# Autodesk Inventor assembly: Blue Alliance Bucket
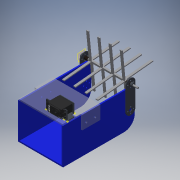
[picture p0: Inventor's stored thumbnail of the model, 180x180]
Saved by Autodesk Inventor 2016 (Build 200138000, 138)
## iProperties
Created: 2015-12-16
Part Number: Blue Alliance Bucket
Document SubType Name: Assembly
Designer: TimB
Author: TimB
## Documents named in this file (10)
- C:\Users\tbloo\Documents\GitHub\phi_robotics\3d-models\FTC_Tetrix_KOP_Block_Party\Tim Bloot Designs\JAr JaR Bot\Blue Alliance Bucket.iam
- C:\Users\tbloo\Documents\GitHub\phi_robotics\3d-models\FTC_Tetrix_KOP_Block_Party\Tim Bloot Designs\JAr JaR Bot\Bucket - BlueA.ipt
- C:\Users\tbloo\Documents\GitHub\phi_robotics\3d-models\FTC_Tetrix_KOP_Block_Party\Tetrix_Kit_FTC\Autodesk Inventor Files\tetrix_servo_mount.ipt
- C:\Users\tbloo\Documents\GitHub\phi_robotics\3d-models\FTC_Tetrix_KOP_Block_Party\Tetrix_Kit_FTC\Autodesk Inventor Files\tetrix_739061_2012.ipt
- C:\Users\tbloo\Documents\GitHub\phi_robotics\3d-models\FTC_Tetrix_KOP_Block_Party\Tim Bloot Designs\JAr JaR Bot\Bucket -  Top.ipt
- C:\Users\tbloo\Documents\GitHub\phi_robotics\3d-models\FTC_Tetrix_KOP_Block_Party\Tetrix_Kit_FTC\Autodesk Inventor Files\tetrix_servo_body.ipt
- C:\Users\tbloo\Documents\GitHub\phi_robotics\3d-models\FTC_Tetrix_KOP_Block_Party\Tetrix_Kit_FTC\Autodesk Inventor Files\tetrix_739092_2012.iam
- C:\Users\tbloo\Documents\GitHub\phi_robotics\3d-models\FTC_Tetrix_KOP_Block_Party\Tetrix_Kit_FTC\Autodesk Inventor Files\tetrix_bushing.ipt
- C:\Users\tbloo\Documents\GitHub\phi_robotics\3d-models\FTC_Tetrix_KOP_Block_Party\Tim Bloot Designs\JAr JaR Bot\Bucket - 4 Rake.iam
- C:\Users\tbloo\Documents\GitHub\phi_robotics\3d-models\FTC_Tetrix_KOP_Block_Party\Tim Bloot Designs\JAr JaR Bot\Bucket - Axle.ipt
## Components (12 placed, 9 different names)
1. Bucket - BlueA:1 — Rigid:2, Rigid:3, Rigid:4
2. tetrix_739061_2012:1 — Rigid:2, Rotational:3
3. tetrix_739061_2012:2 — Rigid:3, Rotational:4
4. Bucket -  Top:1 — Rigid:4, Rigid:9
5. tetrix_739092_2012:1 [sub-assembly]
6. tetrix_739092_2012:2 [sub-assembly] — Rotational:5, Rigid:6
7. tetrix_bushing:1 — Rotational:3
8. Bucket - 4 Rake:1 [sub-assembly] — Rigid:7
9. tetrix_bushing:2 — Rotational:4, Rotational:5
10. Bucket - Axle:1 — Rigid:6, Rigid:7
11. tetrix_servo_mount:1 — Rigid:8, Rigid:9
12. tetrix_servo_body:2 — Rigid:8
## Relationships (10: WeldJoint 7, RevoluteJoint 3)
- Rigid:2 [WeldJoint]: Bucket - BlueA:1 ↔ tetrix_739061_2012:1
- Rigid:3 [WeldJoint]: Bucket - BlueA:1 ↔ tetrix_739061_2012:2
- Rigid:4 [WeldJoint]: Bucket - BlueA:1 ↔ Bucket -  Top:1
- Rotational:3 [RevoluteJoint]: tetrix_739061_2012:1 ↔ tetrix_bushing:1
- Rotational:4 [RevoluteJoint]: tetrix_739061_2012:2 ↔ tetrix_bushing:2
- Rotational:5 [RevoluteJoint]: tetrix_739092_2012:2 ↔ tetrix_bushing:2
- Rigid:6 [WeldJoint]: tetrix_739092_2012:2 ↔ Bucket - Axle:1
- Rigid:7 [WeldJoint] (-10 mm): Bucket - 4 Rake:1 ↔ Bucket - Axle:1
- Rigid:8 [WeldJoint]: tetrix_servo_mount:1 ↔ tetrix_servo_body:2
- Rigid:9 [WeldJoint]: Bucket -  Top:1 ↔ tetrix_servo_mount:1
